# Autodesk Inventor assembly: iceTubeClockAssembly
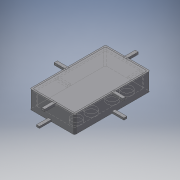
[picture p0: Inventor's stored thumbnail of the model, 180x180]
Saved by Autodesk Inventor 2016 (Build 200138000, 138)
## iProperties
Created: 2016-04-01
Part Number: iceTubeClockAssembly
Document SubType Name: Assembly
Designer: boztalay
Author: boztalay
## Documents named in this file (3)
- \\engin-labs.m.storage.umich.edu\boztalay\iceTubeClockAssemblyRevised.iam
- \\engin-labs.m.storage.umich.edu\boztalay\iceTubeClockBaseRevised.ipt
- \\engin-labs.m.storage.umich.edu\boztalay\iceTubeClockTopRevised.ipt
## Components (2 placed, 2 different names)
1. iceTubeClockBaseRevised:1 — Mate:1, Mate:2, Mate:3
2. iceTubeClockTopRevised:1 — Mate:1, Mate:2, Mate:3
## Relationships (3: Mate 3)
- Mate:1: iceTubeClockBaseRevised:1 ↔ iceTubeClockTopRevised:1
- Mate:2: iceTubeClockBaseRevised:1 ↔ iceTubeClockTopRevised:1
- Mate:3: iceTubeClockBaseRevised:1 ↔ iceTubeClockTopRevised:1
